# Autodesk Inventor assembly: Assembly1
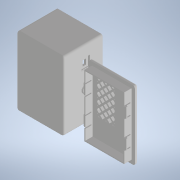
[picture p0: Inventor's stored thumbnail of the model, 180x180]
Saved by Autodesk Inventor 2022.6 (Build 266554010, 554A)
## iProperties
Created: 2025-05-14
Part Number: Assembly1
Document SubType Name: Assembly
Designer: khinm
Author: khinm
## Documents named in this file (3)
- C:\Users\khinm\Downloads\CAD\design_v1.1\Assembly1.iam
- C:\Users\khinm\Downloads\CAD\design_v1.1\Part_A1.ipt
- C:\Users\khinm\Downloads\CAD\design_v1.1\Part_A2.ipt
## Components (2 placed, 2 different names)
1. Part_A1:1 — Mate:1, Mate:2
2. Part_A2:1 — Mate:1, Mate:2
## Relationships (2: Mate 2)
- Mate:1: Part_A1:1 ↔ Part_A2:1
- Mate:2: Part_A1:1 ↔ Part_A2:1
